# Autodesk Inventor assembly: Cybergear_Arm
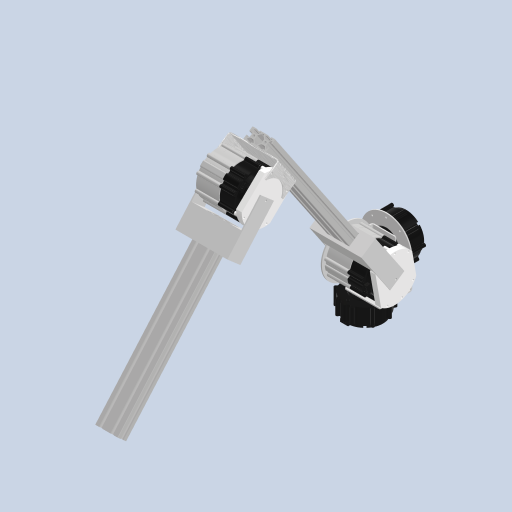
[picture p0: Inventor's stored thumbnail of the model, 512x512]
Saved by Autodesk Inventor 2023 (Build 270158000, 158)
## iProperties
Created: 2024-08-27
Part Number: Cybergear_Arm
Document SubType Name: Assembly
Designer: kiyo
Author: kiyo
## Documents named in this file (9)
- D:\GitHub\inventor\OfficeRobot\Manipulator\Cybergear_Arm.iam
- D:\GitHub\inventor\OfficeRobot\ReadyMade\CyberGear\CyberGearmotor.iam
- D:\GitHub\inventor\OfficeRobot\Manipulator\serbo_bracket.ipt
- D:\GitHub\inventor\OfficeRobot\Manipulator\serbo_bracket2.ipt
- D:\GitHub\inventor\OfficeRobot\ReadyMade\CyberGear\PlanetaryGear-3_5xReducer\PlanetaryGear-3_5xReducer.iam
- D:\GitHub\inventor\OfficeRobot\Manipulator\Jig\Jig1.ipt
- D:\GitHub\inventor\OfficeRobot\Manipulator\servo_arm.ipt
- D:\GitHub\inventor\OfficeRobot\ReadyMade\HFSB5-2040-300.ipt
- D:\GitHub\inventor\OfficeRobot\Manipulator\frame_arm.ipt
## Components (15 placed, 8 different names)
1. CyberGearmotor:1 [sub-assembly] — 角度:5, 角度:6, 挿入:17, 挿入:18
2. CyberGearmotor:2 [sub-assembly] — 挿入:25, 挿入:26, 挿入:27, 挿入:28
3. CyberGearmotor:3 [sub-assembly] — 挿入:19, 角度:7, 挿入:20, 挿入:21
4. serbo_bracket:1 — 挿入:17, 挿入:18, 挿入:19
5. serbo_bracket2:1 — 挿入:20, 挿入:21, 挿入:29, 挿入:30
6. PlanetaryGear-3_5xReducer:1 [sub-assembly] — 挿入:25, 挿入:26, 挿入:29, 挿入:30, 挿入:31
7. Jig1:1 — 挿入:27, 挿入:28
8. HFSB5-2040-300:1 — メイト:1, メイト:2, フラッシュ:1, メイト:3, フラッシュ:2, フラッシュ:3
9. frame_arm:1 — 挿入:31, メイト:1, メイト:2, フラッシュ:1
10. CyberGearmotor:4 [sub-assembly]
11. PlanetaryGear-3_5xReducer:2 [sub-assembly] — 挿入:38
12. Jig1:2 — 挿入:36, 挿入:37
13. servo_arm:1 — メイト:3, フラッシュ:2, フラッシュ:3, 挿入:36, 挿入:37
14. HFSB5-2040-300:2
15. frame_arm:2 — 挿入:38
## Relationships (31: Insert 19, Mate 5, Flush 4, Angle 3)
- 角度:5 [Angle] (0 deg): CyberGearmotor:1
- 角度:6 [Angle] (0 deg): CyberGearmotor:1
- 挿入:17 [Insert]: CyberGearmotor:1 ↔ serbo_bracket:1
- 挿入:18 [Insert]: CyberGearmotor:1 ↔ serbo_bracket:1
- 挿入:19 [Insert]: CyberGearmotor:3 ↔ serbo_bracket:1
- 角度:7 [Angle] (90 deg): CyberGearmotor:3
- 挿入:20 [Insert]: CyberGearmotor:3 ↔ serbo_bracket2:1
- 挿入:21 [Insert]: CyberGearmotor:3 ↔ serbo_bracket2:1
- 挿入:25 [Insert]: CyberGearmotor:2 ↔ PlanetaryGear-3_5xReducer:1
- 挿入:26 [Insert]: CyberGearmotor:2 ↔ PlanetaryGear-3_5xReducer:1
- 挿入:27 [Insert]: CyberGearmotor:2 ↔ Jig1:1
- 挿入:28 [Insert]: CyberGearmotor:2 ↔ Jig1:1
- 挿入:29 [Insert]: serbo_bracket2:1 ↔ PlanetaryGear-3_5xReducer:1
- 挿入:30 [Insert]: serbo_bracket2:1 ↔ PlanetaryGear-3_5xReducer:1
- 挿入:31 [Insert]: PlanetaryGear-3_5xReducer:1 ↔ frame_arm:1
- メイト:1 [Mate] (0.25 mm): HFSB5-2040-300:1 ↔ frame_arm:1
- メイト:2 [Mate] (0.25 mm): HFSB5-2040-300:1 ↔ frame_arm:1
- フラッシュ:1 [Flush]: HFSB5-2040-300:1 ↔ frame_arm:1
- [Insert]: CyberGearmotor:4 ↔ PlanetaryGear-3_5xReducer:2
- [Insert]: CyberGearmotor:4 ↔ PlanetaryGear-3_5xReducer:2
- [Insert]: CyberGearmotor:4 ↔ Jig1:2
- [Insert]: CyberGearmotor:4 ↔ Jig1:2
- メイト:3 [Mate]: HFSB5-2040-300:1 ↔ servo_arm:1
- フラッシュ:2 [Flush]: HFSB5-2040-300:1 ↔ servo_arm:1
- フラッシュ:3 [Flush] (-24 mm): HFSB5-2040-300:1 ↔ servo_arm:1
- 挿入:36 [Insert]: Jig1:2 ↔ servo_arm:1
- 挿入:37 [Insert]: Jig1:2 ↔ servo_arm:1
- [Mate] (0.25 mm): HFSB5-2040-300:2 ↔ frame_arm:2
- [Mate] (0.25 mm): HFSB5-2040-300:2 ↔ frame_arm:2
- [Flush]: HFSB5-2040-300:2 ↔ frame_arm:2
- 挿入:38 [Insert]: PlanetaryGear-3_5xReducer:2 ↔ frame_arm:2
## Named parameters: d71_d58 = 0 mm, d72_d55 = 0 mm, d73_d56 = 0 mm, d74_d57 = 0 mm, d81_d68 = 0.25 mm, d82_d69 = 0.25 mm, d83_d70 = 0 mm
